# Autodesk Inventor assembly: 800-BATTERY-PACK
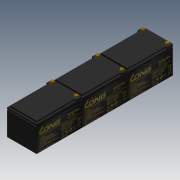
[picture p0: Inventor's stored thumbnail of the model, 180x180]
Saved by Autodesk Inventor 2018.2 (Build 222227000, 227)
## iProperties
Manager: feesmrt
Company: FRANCOR
Part Number: 800-BATTERY-PACK
Project: Rescue Robot
Cost Center: -
Material: Generisch
Document SubType Name: Assembly
Designer: feesmrt
Engineer: feesmrt
Authority: feesmrt
Description: Battery Pack ASM
Stock Number: 800-BATTERY-PACK
Subject: Rescue Robot
Author: feesmrt
Revision Number: 1
Title: Battery Pack ASM
## Documents named in this file (2)
- D:\Programmierung\FRANC0R\CAD\02-Rocker-Bogie-Robot\800-ELECTRONICS\800-BATTERY-PACK.iam
- D:\Programmierung\FRANC0R\CAD\02-Rocker-Bogie-Robot\800-ELECTRONICS\800-10-ELECTRONICS-BATTERY\800-10-ELECTRONICS-BATTERY-12V-12Ah.ipt
## Components (3 placed, 1 different names)
1. 800-10-ELECTRONICS-BATTERY-12V-12Ah:1 — Fluchtend:1, Fluchtend:2, Fluchtend:3, Fluchtend:4, Passend:1, Passend:2
2. 800-10-ELECTRONICS-BATTERY-12V-12Ah:2 — Fluchtend:1, Fluchtend:2, Passend:2
3. 800-10-ELECTRONICS-BATTERY-12V-12Ah:3 — Fluchtend:3, Fluchtend:4, Passend:1
## Relationships (6: Flush 4, Mate 2)
- Fluchtend:1 [Flush]: 800-10-ELECTRONICS-BATTERY-12V-12Ah:1 ↔ 800-10-ELECTRONICS-BATTERY-12V-12Ah:2
- Fluchtend:2 [Flush]: 800-10-ELECTRONICS-BATTERY-12V-12Ah:1 ↔ 800-10-ELECTRONICS-BATTERY-12V-12Ah:2
- Fluchtend:3 [Flush]: 800-10-ELECTRONICS-BATTERY-12V-12Ah:1 ↔ 800-10-ELECTRONICS-BATTERY-12V-12Ah:3
- Fluchtend:4 [Flush]: 800-10-ELECTRONICS-BATTERY-12V-12Ah:1 ↔ 800-10-ELECTRONICS-BATTERY-12V-12Ah:3
- Passend:1 [Mate]: 800-10-ELECTRONICS-BATTERY-12V-12Ah:1 ↔ 800-10-ELECTRONICS-BATTERY-12V-12Ah:3
- Passend:2 [Mate]: 800-10-ELECTRONICS-BATTERY-12V-12Ah:1 ↔ 800-10-ELECTRONICS-BATTERY-12V-12Ah:2
## Named parameters: Battery_Distance = 2.5 mm
